# Autodesk Inventor assembly: robot_polea
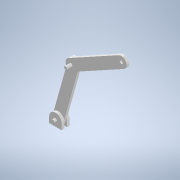
[picture p0: Inventor's stored thumbnail of the model, 180x180]
Saved by Autodesk Inventor 2021 (Build 250183000, 183)
## iProperties
Created: 2022-01-22
Part Number: robot_polea
Document SubType Name: Assembly
Designer: Yeison
Author: Yeison
## Documents named in this file (4)
- C:\Users\Yeison\Documents\GitHub\Servomecanismos\Modelo 2021\robot_polea.iam
- C:\Users\Yeison\Documents\GitHub\Servomecanismos\Modelo 2021\Soporte.ipt
- C:\Users\Yeison\Documents\GitHub\Servomecanismos\Modelo 2021\pin2.ipt
- C:\Users\Yeison\Documents\GitHub\Servomecanismos\Modelo 2021\Eslabon.ipt
## Components (5 placed, 3 different names)
1. Soporte:1 — Rotational:1, Rotational:2
2. pin2:1 — Rotational:1
3. Eslabon:1 — Rotational:2, Rotational:3
4. pin2:2 — Rotational:3, Rigid:1
5. Eslabon:2 — Rigid:1
## Relationships (4: RevoluteJoint 3, WeldJoint 1)
- Rotational:1 [RevoluteJoint]: Soporte:1 ↔ pin2:1
- Rotational:2 [RevoluteJoint]: Soporte:1 ↔ Eslabon:1
- Rotational:3 [RevoluteJoint]: Eslabon:1 ↔ pin2:2
- Rigid:1 [WeldJoint]: pin2:2 ↔ Eslabon:2
